# Autodesk Inventor assembly: double bearing
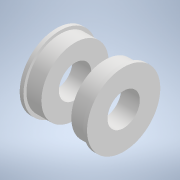
[picture p0: Inventor's stored thumbnail of the model, 180x180]
Saved by Autodesk Inventor 2020 (Build 240168000, 168)
## iProperties
Created: 2020-02-03
Part Number: double bearing
Document SubType Name: Assembly
Designer: aidan
Author: aidan
## Documents named in this file (2)
- C:\Users\aidan\Desktop\T3 Robotics\CAD\Generic and Stock\double bearing.iam
- C:\Users\aidan\Desktop\T3 Robotics\CAD\Bearing for THUNDER.ipt
## Components (2 placed, 1 different names)
1. Bearing for THUNDER:1 — Mate:1, Mate:2
2. Bearing for THUNDER:2 — Mate:1, Mate:2
## Relationships (2: Mate 2)
- Mate:1: Bearing for THUNDER:1 ↔ Bearing for THUNDER:2
- Mate:2 (25.4 mm): Bearing for THUNDER:1 ↔ Bearing for THUNDER:2
